# Autodesk Inventor assembly: modelo cad brazo
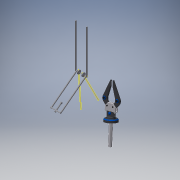
[picture p0: Inventor's stored thumbnail of the model, 180x180]
Saved by Autodesk Inventor 2016 (Build 200138000, 138)
## iProperties
Created: 2016-07-27
Part Number: modelo cad brazo
Document SubType Name: Assembly
Designer: Admin
Author: Admin
## Documents named in this file (11)
- C:\Users\Admin\Documents\diseños autodesk dimer\modelo cad\modelo cad brazo.iam
- C:\Users\Admin\Documents\diseños autodesk dimer\modelo cad\modelo cad brazo.ipt
- C:\Users\Admin\Documents\diseños autodesk dimer\modelo cad\antebrazo.ipt
- C:\Users\Admin\Documents\diseños autodesk dimer\modelo cad\rodamientos medio.ipt
- C:\Users\Admin\Documents\diseños autodesk dimer\modelo cad\barra muñeca.ipt
- C:\Users\Admin\Documents\diseños autodesk dimer\modelo cad\muñeca eje.ipt
- C:\Users\Admin\Documents\diseños autodesk dimer\modelo cad\enganche eje muñeca.ipt
- C:\Users\Admin\Downloads\robotic-arm--3\Robotic Arm\Gripper.ipt
- C:\Users\Admin\Downloads\robotic-arm--3\Robotic Arm\Finger.ipt
- C:\Users\Admin\Downloads\robotic-arm--3\Robotic Arm\Holder.ipt
- C:\Users\Admin\Downloads\robotic-arm--3\Robotic Arm\Pin.ipt
## Components (12 placed, 10 different names)
1. modelo cad brazo:1 — Mate:1, Mate:2
2. antebrazo:1 — Mate:1, Mate:2, Mate:3, Mate:4, Mate:5, Mate:6, Flush:1
3. rodamientos medio:1 — Mate:3
4. rodamientos medio:2 — Mate:4
5. barra muñeca:1 — Mate:5, Mate:6, Flush:1, Mate:7, Flush:2, Tangent:1
6. muñeca eje:1 — Tangent:1, Mate:8
7. enganche eje muñeca:1 — Mate:7, Flush:2, Mate:8
8. Gripper:1
9. Finger:1
10. Finger:2
11. Holder:1
12. Pin:1
## Relationships (19: Mate 16, Flush 2, Tangent 1)
- Mate:1 (0.75 mm): modelo cad brazo:1 ↔ antebrazo:1
- Mate:2: modelo cad brazo:1 ↔ antebrazo:1
- Mate:3: antebrazo:1 ↔ rodamientos medio:1
- Mate:4: antebrazo:1 ↔ rodamientos medio:2
- Mate:5 (-10 mm): antebrazo:1 ↔ barra muñeca:1
- Mate:6 (-22 mm): antebrazo:1 ↔ barra muñeca:1
- Flush:1: antebrazo:1 ↔ barra muñeca:1
- Mate:7: barra muñeca:1 ↔ enganche eje muñeca:1
- Flush:2: barra muñeca:1 ↔ enganche eje muñeca:1
- Tangent:1: barra muñeca:1 ↔ muñeca eje:1
- Mate:8 (-80 mm): muñeca eje:1 ↔ enganche eje muñeca:1
- [Mate]: Gripper:1 ↔ Holder:1
- [Mate] (2.5 mm): Gripper:1 ↔ Holder:1
- [Mate]: Finger:2 ↔ Holder:1
- [Mate]: Finger:1 ↔ Holder:1
- [Mate]: Finger:1 ↔ Holder:1
- [Mate]: Finger:2 ↔ Holder:1
- [Mate]: Holder:1 ↔ Pin:1
- [Mate] (-50 mm): Gripper:1 ↔ Pin:1
